# Autodesk Inventor assembly: TestSoporte
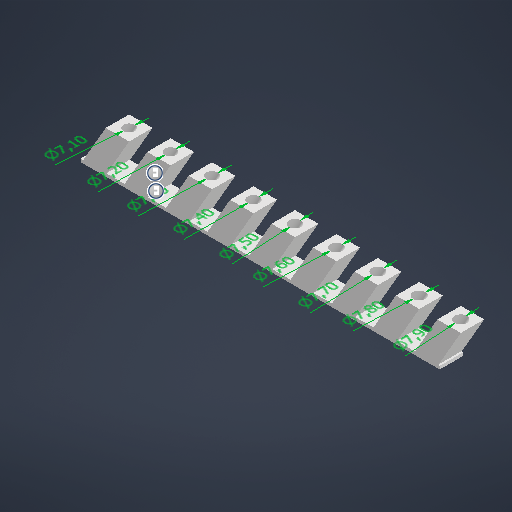
[picture p0: Inventor's stored thumbnail of the model, 512x512]
Saved by Autodesk Inventor 2026.1 (Build 301233000, 233)
## iProperties
Created: 2025-10-12
Part Number: TestSoporte
Document SubType Name: Assembly
Designer: tito.luyo
Author: tito.luyo
## Documents named in this file (11)
- C:\work\verticalparking\diseno3d\Testing\TestSoporte.iam
- C:\work\verticalparking\diseno3d\Testing\TestSoporte - Copy.ipt
- C:\work\verticalparking\diseno3d\Testing\TestSoporte - Copy (2).ipt
- C:\work\verticalparking\diseno3d\Testing\TestSoporte - Copy (3).ipt
- C:\work\verticalparking\diseno3d\Testing\TestSoporte - Copy (4).ipt
- C:\work\verticalparking\diseno3d\Testing\TestSoporte - Copy (5).ipt
- C:\work\verticalparking\diseno3d\Testing\TestSoporte - Copy (6).ipt
- C:\work\verticalparking\diseno3d\Testing\TestSoporte - Copy (7).ipt
- C:\work\verticalparking\diseno3d\Testing\TestSoporte - Copy (8).ipt
- C:\work\verticalparking\diseno3d\Testing\TestSoporte - Copy (9).ipt
- C:\work\verticalparking\diseno3d\Testing\TestBaseSoportes.ipt
## Components (10 placed, 10 different names)
1. TestSoporte - Copy:1 — Flush:1, Flush:2, Mate:1, Mate:9, Flush:17
2. TestSoporte - Copy (2):1 — Flush:1, Flush:2, Mate:1, Flush:3, Flush:4, Mate:2
3. TestSoporte - Copy (3):1 — Flush:3, Flush:4, Mate:2, Flush:5, Flush:6, Mate:3
4. TestSoporte - Copy (4):1 — Flush:5, Flush:6, Mate:3, Flush:7, Flush:8, Mate:4
5. TestSoporte - Copy (5):1 — Flush:7, Flush:8, Mate:4, Mate:5, Flush:9, Flush:10
6. TestSoporte - Copy (6):1 — Mate:5, Flush:9, Flush:10, Mate:6, Flush:11, Flush:12
7. TestSoporte - Copy (7):1 — Mate:6, Flush:11, Flush:12, Mate:7, Flush:13, Flush:14
8. TestSoporte - Copy (8):1 — Mate:7, Flush:13, Flush:14, Mate:8, Flush:15, Flush:16
9. TestSoporte - Copy (9):1 — Mate:8, Flush:15, Flush:16
10. TestBaseSoportes:1 — Mate:9, Flush:17
## Relationships (26: Flush 17, Mate 9)
- Flush:1: TestSoporte - Copy:1 ↔ TestSoporte - Copy (2):1
- Flush:2: TestSoporte - Copy:1 ↔ TestSoporte - Copy (2):1
- Mate:1 (10 mm): TestSoporte - Copy:1 ↔ TestSoporte - Copy (2):1
- Flush:3: TestSoporte - Copy (2):1 ↔ TestSoporte - Copy (3):1
- Flush:4: TestSoporte - Copy (2):1 ↔ TestSoporte - Copy (3):1
- Mate:2 (10 mm): TestSoporte - Copy (2):1 ↔ TestSoporte - Copy (3):1
- Flush:5: TestSoporte - Copy (3):1 ↔ TestSoporte - Copy (4):1
- Flush:6: TestSoporte - Copy (3):1 ↔ TestSoporte - Copy (4):1
- Mate:3 (10 mm): TestSoporte - Copy (3):1 ↔ TestSoporte - Copy (4):1
- Flush:7: TestSoporte - Copy (4):1 ↔ TestSoporte - Copy (5):1
- Flush:8: TestSoporte - Copy (4):1 ↔ TestSoporte - Copy (5):1
- Mate:4 (10 mm): TestSoporte - Copy (4):1 ↔ TestSoporte - Copy (5):1
- Mate:5 (10 mm): TestSoporte - Copy (5):1 ↔ TestSoporte - Copy (6):1
- Flush:9: TestSoporte - Copy (5):1 ↔ TestSoporte - Copy (6):1
- Flush:10: TestSoporte - Copy (5):1 ↔ TestSoporte - Copy (6):1
- Mate:6 (10 mm): TestSoporte - Copy (6):1 ↔ TestSoporte - Copy (7):1
- Flush:11: TestSoporte - Copy (6):1 ↔ TestSoporte - Copy (7):1
- Flush:12: TestSoporte - Copy (6):1 ↔ TestSoporte - Copy (7):1
- Mate:7 (10 mm): TestSoporte - Copy (7):1 ↔ TestSoporte - Copy (8):1
- Flush:13: TestSoporte - Copy (7):1 ↔ TestSoporte - Copy (8):1
- Flush:14: TestSoporte - Copy (7):1 ↔ TestSoporte - Copy (8):1
- Mate:8 (10 mm): TestSoporte - Copy (8):1 ↔ TestSoporte - Copy (9):1
- Flush:15: TestSoporte - Copy (8):1 ↔ TestSoporte - Copy (9):1
- Flush:16: TestSoporte - Copy (8):1 ↔ TestSoporte - Copy (9):1
- Mate:9: TestSoporte - Copy:1 ↔ TestBaseSoportes:1
- Flush:17: TestSoporte - Copy:1 ↔ TestBaseSoportes:1
